# Autodesk Inventor assembly: VersaPlanetary_v2_Single_Stage_10_1_with_RS_550
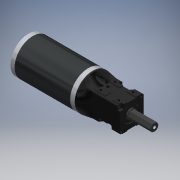
[picture p0: Inventor's stored thumbnail of the model, 180x180]
Saved by Autodesk Inventor 2017 SP1 (Build 210196100, 196)
## iProperties
Created: 2016-10-31
Part Number: VersaPlanetary_v2_Single_Stage_10_1_with_RS_550
Description: STEP AP214
Document SubType Name: Assembly
Designer: Ben
Sending System: SolidWorks 2016
Preprocessor: SwSTEP 2.0
Title: 217-4973_1stage_550.STEP
Revision Number: ANY
## Documents named in this file (14)
- C:\Users\Ben\Desktop\Projects\2018 Robot\Cube Lift\Drive motor\VersaPlanetary_v2_Single_Stage_10_1_with_RS_550.iam
- C:\Users\Ben\Desktop\Projects\2018 Robot\Cube Lift\Drive motor\217-2625-026 Rev1.ipt
- C:\Users\Ben\Desktop\Projects\2018 Robot\Cube Lift\Drive motor\217-2742-001 Rev4.ipt
- C:\Users\Ben\Desktop\Projects\2018 Robot\Cube Lift\Drive motor\217-2625-017 Rev1_9714K61.ipt
- C:\Users\Ben\Desktop\Projects\2018 Robot\Cube Lift\Drive motor\217-2625-003 Rev1.ipt
- C:\Users\Ben\Desktop\Projects\2018 Robot\Cube Lift\Drive motor\217-2625-018 Rev1_98541A410.ipt
- C:\Users\Ben\Desktop\Projects\2018 Robot\Cube Lift\Drive motor\217-2625-025 Rev1.ipt
- C:\Users\Ben\Desktop\Projects\2018 Robot\Cube Lift\Drive motor\217-2820 Rev1_Public.iam
- C:\Users\Ben\Desktop\Projects\2018 Robot\Cube Lift\Drive motor\217-2816-001 Rev1.ipt
- C:\Users\Ben\Desktop\Projects\2018 Robot\Cube Lift\Drive motor\217-4649-001 Rev1.ipt
- C:\Users\Ben\Desktop\Projects\2018 Robot\Cube Lift\Drive motor\217-4649-007 Rev1_94105A824.ipt
- C:\Users\Ben\Desktop\Projects\2018 Robot\Cube Lift\Drive motor\217-2625-012 Rev1.ipt
- C:\Users\Ben\Desktop\Projects\2018 Robot\Cube Lift\Drive motor\VersaPlanetary_CIM_Adapter_217-4018.ipt
- C:\Users\Ben\Desktop\Projects\2018 Robot\Cube Lift\Drive motor\am-0255+2.5inch+CIM+Motor.ipt
## Components (14 placed, 14 different names)
1. 217-2625-026 Rev1_1
2. 217-2742-001 Rev4_2
3. 217-2742-001 Rev4_3
4. 217-2625-017 Rev1_9714K61_4
5. 217-2625-003 Rev1_5
6. 217-2625-018 Rev1_98541A410_6
7. 217-2625-025 Rev1_9 — Insert:1, Mate:1
8. 217-2820 Rev1_Public_16 [sub-assembly]
9. 217-2816-001 Rev1_17
10. 217-4649-001 Rev1_18
11. 217-4649-007 Rev1_94105A824_19
12. 217-2625-012 Rev1_20
13. VersaPlanetary_CIM_Adapter_217-4018:1 — Insert:1, Mate:1, Insert:2
14. am-0255+2.5inch+CIM+Motor:1 — Insert:2
## Relationships (3: Insert 2, Mate 1)
- Insert:1: 217-2625-025 Rev1_9 ↔ VersaPlanetary_CIM_Adapter_217-4018:1
- Mate:1: 217-2625-025 Rev1_9 ↔ VersaPlanetary_CIM_Adapter_217-4018:1
- Insert:2: VersaPlanetary_CIM_Adapter_217-4018:1 ↔ am-0255+2.5inch+CIM+Motor:1
